# Autodesk Inventor assembly: Modelado de eqilibrador
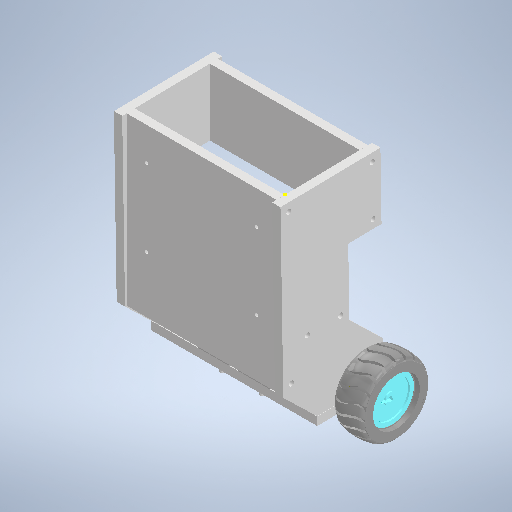
[picture p0: Inventor's stored thumbnail of the model, 512x512]
Saved by Autodesk Inventor 2025.2 (Build 292293000, 293)
## iProperties
Created: 2025-01-27
Part Number: Modelado de eqilibrador
Document SubType Name: Assembly
Designer: alex
Author: alex
## Documents named in this file (10)
- C:\Users\alex\Documents\Git\Control\Proyecto\Modelado de eqilibrador.iam
- C:\Users\alex\Documents\Git\Control\Proyecto\Base.ipt
- C:\Users\alex\Documents\Git\Control\Proyecto\Atras.ipt
- C:\Users\alex\Documents\Git\Control\Proyecto\Lateral.ipt
- C:\Users\alex\Documents\Git\Control\Proyecto\Interno.ipt
- C:\Users\alex\Documents\Git\Control\Proyecto\Frontal.ipt
- C:\Users\alex\Documents\Git\Control\Proyecto\N20 Motor.ipt
- C:\Users\alex\Documents\Git\Control\Proyecto\CR123A  Battery Holder\CR123A  Battery Holder\CR123A  Battery Holder.ipt
- C:\Users\alex\Desktop\esp8266-balancing-robot-1.snapshot.1\resources\Carte proto 7x5\Carte proto 7x5\Carte proto 7x5.ipt
- C:\Users\alex\Desktop\esp8266-balancing-robot-1.snapshot.1\resources\RC wheel\RC wheel\RC wheel.iam
## Components (12 placed, 9 different names)
1. Lateral:1 — Insertar:1, Coincidencia:1, Insertar:3
2. Atras:1 — Insertar:1, Insertar:2, Insertar:10
3. Lateral:2 — Insertar:2, Coincidencia:2, Coincidencia:3, Insertar:4
4. Base:1 — Coincidencia:1, Coincidencia:2, Insertar:5, Insertar:6, Insertar:7, Insertar:8, Insertar:9
5. Frontal:1 — Coincidencia:3, Insertar:3
6. Interno:1 — Insertar:4
7. N20 Motor:1 — Insertar:5, Insertar:6, De rotación:1
8. N20 Motor:2 — Insertar:7, Insertar:8, De rotación:2
9. CR123A  Battery Holder:1 — Insertar:9
10. Carte proto 7x5:1 — Insertar:10
11. RC wheel:1 [sub-assembly] — De rotación:2
12. RC wheel:2 [sub-assembly] — De rotación:1
## Relationships (15: Insert 10, Mate 3, RevoluteJoint 2)
- Insertar:1: Lateral:1 ↔ Atras:1
- Insertar:2: Atras:1 ↔ Lateral:2
- Coincidencia:1 [Mate]: Lateral:1 ↔ Base:1
- Coincidencia:2 [Mate]: Lateral:2 ↔ Base:1
- Coincidencia:3 [Mate]: Lateral:2 ↔ Frontal:1
- Insertar:3: Lateral:1 ↔ Frontal:1
- Insertar:4: Lateral:2 ↔ Interno:1
- Insertar:5: Base:1 ↔ N20 Motor:1
- Insertar:6: Base:1 ↔ N20 Motor:1
- Insertar:7: Base:1 ↔ N20 Motor:2
- Insertar:8: Base:1 ↔ N20 Motor:2
- Insertar:9: Base:1 ↔ CR123A  Battery Holder:1
- Insertar:10: Atras:1 ↔ Carte proto 7x5:1
- De rotación:1 [RevoluteJoint]: N20 Motor:1 ↔ RC wheel:2
- De rotación:2 [RevoluteJoint]: N20 Motor:2 ↔ RC wheel:1
